# Autodesk Inventor assembly: Layout
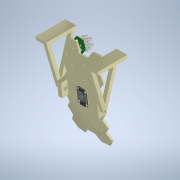
[picture p0: Inventor's stored thumbnail of the model, 180x180]
Saved by Autodesk Inventor 2022 (Build 260153070, 153G)
## iProperties
Created: 2021-11-18
Part Number: Layout
Document SubType Name: Assembly
Designer: Eric
Author: Eric
## Documents named in this file (5)
- D:\MyRepos\IRheating\3dModels\Layout.iam
- D:\MyRepos\IRheating\KiCAD\sevenLEDboard.ipt
- D:\MyRepos\IRheating\3dModels\ArrayBracket.ipt
- D:\MyRepos\IRheating\3dModels\Camara_MLX90640.ipt
- D:\MyRepos\IRheating\3dModels\ArrayBracketSupport.ipt
## Components (5 placed, 4 different names)
1. sevenLEDboard:1 — Mate:1, Angle:1, Mate:2
2. ArrayBracket:1 — Mate:1, Angle:1, Insert:2, Mate:2, Angle:3, Insert:4, Insert:5
3. Camara_MLX90640:1 — Insert:2, Angle:3
4. ArrayBracketSupport:1 — Angle:2, Mate:3, Mate:4, Mate:5, Insert:5
5. ArrayBracketSupport:2 — Angle:2, Insert:4
## Relationships (11: Mate 5, Angle 3, Insert 3)
- Mate:1: sevenLEDboard:1 ↔ ArrayBracket:1
- Angle:1 (0 deg): sevenLEDboard:1 ↔ ArrayBracket:1
- Insert:2: ArrayBracket:1 ↔ Camara_MLX90640:1
- Angle:2 (0 deg): ArrayBracketSupport:1 ↔ ArrayBracketSupport:2
- Mate:2: sevenLEDboard:1 ↔ ArrayBracket:1
- Mate:3: ArrayBracketSupport:1
- Mate:4: ArrayBracketSupport:1
- Mate:5: ArrayBracketSupport:1
- Angle:3 (0 deg): ArrayBracket:1 ↔ Camara_MLX90640:1
- Insert:4: ArrayBracket:1 ↔ ArrayBracketSupport:2
- Insert:5: ArrayBracket:1 ↔ ArrayBracketSupport:1
